# Autodesk Inventor assembly: winch prototype
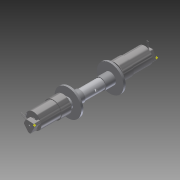
[picture p0: Inventor's stored thumbnail of the model, 180x180]
Saved by Autodesk Inventor 2013 (Build 170138000, 138)
## iProperties
Created: 2013-12-07
Part Number: winch prototype
Document SubType Name: Assembly
Designer: kahohbein
Author: kahohbein
## Documents named in this file (5)
- C:\Users\kahohbein\Documents\GitHub\2013-2014_BlockParty\CAD\Lift\MK2\winch prototype.iam
- C:\Users\kahohbein\Documents\GitHub\2013-2014_BlockParty\CAD\COTSParts\Structural\PVC Spacer 500 Sched 40.ipt
- C:\Users\kahohbein\Documents\GitHub\2013-2014_BlockParty\CAD\COTSParts\Hubs\Hub 8mm key.ipt
- C:\Users\kahohbein\Documents\GitHub\2013-2014_BlockParty\CAD\COTSParts\Tetrix\Tetrix hub - motor.ipt
- C:\Users\kahohbein\Documents\GitHub\2013-2014_BlockParty\CAD\COTSParts\Tetrix\Tetrix motor.ipt
## Components (7 placed, 4 different names)
1. PVC Spacer 500 Sched 40:1 — Mate:1, Mate:2, Mate:3, Mate:4
2. Hub 500key:1 — Mate:1, Mate:2, Mate:5, Mate:6
3. Hub 500key:2 — Mate:3, Mate:4, Mate:7, Mate:8
4. Tetrix motor:1 — Mate:11, Mate:12, Mate:14
5. Tetrix motor:2 — Mate:9, Mate:10, Mate:13
6. Tetrix hub - motor:1 — Mate:5, Mate:6, Mate:11, Mate:12
7. Tetrix hub - motor:2 — Mate:7, Mate:8, Mate:9, Mate:10
## Relationships (14: Mate 14)
- Mate:1: PVC Spacer 500 Sched 40:1 ↔ Hub 500key:1
- Mate:2: PVC Spacer 500 Sched 40:1 ↔ Hub 500key:1
- Mate:3: PVC Spacer 500 Sched 40:1 ↔ Hub 500key:2
- Mate:4: PVC Spacer 500 Sched 40:1 ↔ Hub 500key:2
- Mate:5: Hub 500key:1 ↔ Tetrix hub - motor:1
- Mate:6: Hub 500key:1 ↔ Tetrix hub - motor:1
- Mate:7: Hub 500key:2 ↔ Tetrix hub - motor:2
- Mate:8: Hub 500key:2 ↔ Tetrix hub - motor:2
- Mate:9: Tetrix motor:2 ↔ Tetrix hub - motor:2
- Mate:10: Tetrix motor:2 ↔ Tetrix hub - motor:2
- Mate:11: Tetrix motor:1 ↔ Tetrix hub - motor:1
- Mate:12: Tetrix motor:1 ↔ Tetrix hub - motor:1
- Mate:13: Tetrix motor:2
- Mate:14: Tetrix motor:1
